# Autodesk Inventor assembly: 64아이들러_MIR1
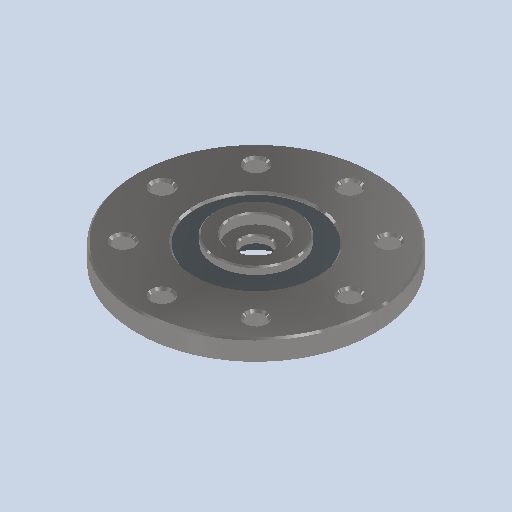
[picture p0: Inventor's stored thumbnail of the model, 512x512]
Saved by Autodesk Inventor 2024.3 (Build 283343000, 343)
## iProperties
Created: 2022-08-09
Part Number: 64아이들러_MIR1
Document SubType Name: Assembly
Designer: 구지현
Mass: 5 g
Surface Area: 21.0198 cm^2
Volume: 1.54681 cm^3
Author: 박지훈
## Documents named in this file (4)
- C:\Users\구지현\Documents\카카오톡 받은 파일\Hardware\ROBOTIS(Inventor 2024 ver.)\아이들러\64아이들러_MIR1.iam
- C:\Users\구지현\Documents\카카오톡 받은 파일\Hardware\ROBOTIS(Inventor 2024 ver.)\아이들러\HN05-i1_MIR1.ipt
- C:\Users\구지현\Documents\카카오톡 받은 파일\Hardware\ROBOTIS(Inventor 2024 ver.)\아이들러\MF128ZZ_MIR1.ipt
- C:\Users\구지현\Documents\카카오톡 받은 파일\Hardware\ROBOTIS(Inventor 2024 ver.)\아이들러\RX64-CAP_MIR1.ipt
## Components (3 placed, 3 different names)
1. HN05-i1_MIR1:1 — 삽입:1
2. MF128ZZ_MIR1:1 — 삽입:1, 삽입:2
3. RX64-CAP_MIR1:1 — 삽입:2
## Relationships (2: Insert 2)
- 삽입:1 [Insert]: HN05-i1_MIR1:1 ↔ MF128ZZ_MIR1:1
- 삽입:2 [Insert]: MF128ZZ_MIR1:1 ↔ RX64-CAP_MIR1:1
